# Autodesk Inventor assembly: Batterie et Support Vertical Réduit
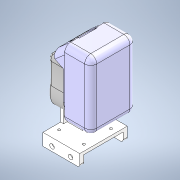
[picture p0: Inventor's stored thumbnail of the model, 180x180]
Saved by Autodesk Inventor 2022 (Build 260153000, 153)
## iProperties
Created: 2021-12-23
Part Number: Batterie et Support Vertical Réduit
Document SubType Name: Assembly
Designer: victo
Author: victo
## Documents named in this file (4)
- C:\Users\victo\Desktop\Documents\ENSTA\Cours ENSTA\2A\PIE\Modélisation\Robot réduit\Batterie et Support Vertical Réduit.iam
- C:\Users\victo\Desktop\Documents\ENSTA\Cours ENSTA\2A\PIE\Modélisation\Modèle - Robot PIE\MAKITA\files\Makita18V_BL1860B.ipt
- C:\Users\victo\Desktop\Documents\ENSTA\Cours ENSTA\2A\PIE\Modélisation\Modèle - Robot PIE\Adaptateur_Makita.ipt
- C:\Users\victo\Desktop\Documents\ENSTA\Cours ENSTA\2A\PIE\Modélisation\Robot réduit\Support_batterie_réduit.ipt
## Components (3 placed, 3 different names)
1. Makita18V_BL1860B:1
2. Adaptateur_Makita:1 — Placage:3, Placage:4, Placage:5
3. Support_batterie_réduit:1 — Placage:3, Placage:4, Placage:5
## Relationships (6: Mate 5, Flush 1)
- [Flush]: Makita18V_BL1860B:1 ↔ Adaptateur_Makita:1
- [Mate]: Makita18V_BL1860B:1 ↔ Adaptateur_Makita:1
- [Mate]: Makita18V_BL1860B:1 ↔ Adaptateur_Makita:1
- Placage:3 [Mate]: Adaptateur_Makita:1 ↔ Support_batterie_réduit:1
- Placage:4 [Mate]: Adaptateur_Makita:1 ↔ Support_batterie_réduit:1
- Placage:5 [Mate]: Adaptateur_Makita:1 ↔ Support_batterie_réduit:1
